# Autodesk Inventor assembly: 26650PACK
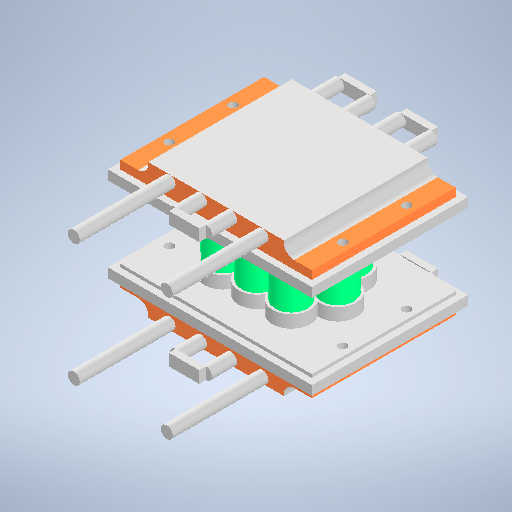
[picture p0: Inventor's stored thumbnail of the model, 512x512]
Saved by Autodesk Inventor 2025.2 (Build 292293000, 293)
## iProperties
Created: 2025-01-16
Part Number: 26650PACK
Document SubType Name: Assembly
Designer: cbast
Author: cbast
## Documents named in this file (6)
- C:\Users\cbast\OneDrive\Documents\26650PACK.iam
- C:\Users\cbast\OneDrive\Documents\26650(Green).ipt
- C:\Users\cbast\OneDrive\Documents\CELLCASE26650.ipt
- C:\Users\cbast\OneDrive\Documents\nickel strip.ipt
- C:\Users\cbast\OneDrive\Documents\cooling plate.ipt
- C:\Users\cbast\OneDrive\Documents\343thermalpad.ipt
## Components (18 placed, 5 different names)
1. 26650(Green):1 — Mate:2, Flush:2
2. 26650(Green):2 — Mate:1, Flush:1
3. 26650(Green):3 — Mate:3, Flush:3
4. 26650(Green):4 — Mate:4, Flush:7, Mate:12, Flush:11
5. 26650(Green):5 — Mate:5, Flush:6
6. 26650(Green):6 — Mate:10, Flush:8
7. 26650(Green):7 — Mate:9, Flush:9
8. 26650(Green):8 — Mate:8, Flush:10
9. 26650(Green):9 — Mate:7, Flush:4, Mate:11
10. 26650(Green):10 — Mate:6, Flush:5
11. CELLCASE26650:1 — Mate:1, Mate:2, Mate:3, Mate:4, Mate:5, Mate:6, Mate:7, Mate:8, Mate:9, Mate:10, Flush:1, Flush:2, Flush:3, Flush:4, Flush:5, Flush:6, Flush:7, Flush:8, Flush:9, Flush:10, Mate:13, Mate:22, Mate:23
12. CELLCASE26650:2 — Mate:11, Mate:12, Flush:11, Mate:15, Mate:18, Mate:19, Mate:20
13. 343thermalpad:1 — Mate:16, Mate:17
14. 343thermalpad:2 — Mate:14, Mate:21
15. nickel strip:1 — Mate:15, Mate:16
16. nickel strip:2 — Mate:13, Mate:14
17. cooling plate:1 — Mate:21, Mate:22, Mate:23
18. cooling plate:2 — Mate:17, Mate:18, Mate:19, Mate:20
## Relationships (34: Mate 23, Flush 11)
- Mate:1: 26650(Green):2 ↔ CELLCASE26650:1
- Mate:2: 26650(Green):1 ↔ CELLCASE26650:1
- Mate:3: 26650(Green):3 ↔ CELLCASE26650:1
- Mate:4: 26650(Green):4 ↔ CELLCASE26650:1
- Mate:5: 26650(Green):5 ↔ CELLCASE26650:1
- Mate:6: 26650(Green):10 ↔ CELLCASE26650:1
- Mate:7: 26650(Green):9 ↔ CELLCASE26650:1
- Mate:8: 26650(Green):8 ↔ CELLCASE26650:1
- Mate:9: 26650(Green):7 ↔ CELLCASE26650:1
- Mate:10: 26650(Green):6 ↔ CELLCASE26650:1
- Flush:1: 26650(Green):2 ↔ CELLCASE26650:1
- Flush:2: 26650(Green):1 ↔ CELLCASE26650:1
- Flush:3: 26650(Green):3 ↔ CELLCASE26650:1
- Flush:4: 26650(Green):9 ↔ CELLCASE26650:1
- Flush:5: 26650(Green):10 ↔ CELLCASE26650:1
- Flush:6: 26650(Green):5 ↔ CELLCASE26650:1
- Flush:7: 26650(Green):4 ↔ CELLCASE26650:1
- Flush:8: 26650(Green):6 ↔ CELLCASE26650:1
- Flush:9: 26650(Green):7 ↔ CELLCASE26650:1
- Flush:10: 26650(Green):8 ↔ CELLCASE26650:1
- Mate:11: 26650(Green):9 ↔ CELLCASE26650:2
- Mate:12: 26650(Green):4 ↔ CELLCASE26650:2
- Flush:11: 26650(Green):4 ↔ CELLCASE26650:2
- Mate:13: CELLCASE26650:1 ↔ nickel strip:2
- Mate:14: 343thermalpad:2 ↔ nickel strip:2
- Mate:15: CELLCASE26650:2 ↔ nickel strip:1
- Mate:16: 343thermalpad:1 ↔ nickel strip:1
- Mate:17: 343thermalpad:1 ↔ cooling plate:2
- Mate:18: CELLCASE26650:2 ↔ cooling plate:2
- Mate:19: CELLCASE26650:2 ↔ cooling plate:2
- Mate:20: CELLCASE26650:2 ↔ cooling plate:2
- Mate:21: 343thermalpad:2 ↔ cooling plate:1
- Mate:22: CELLCASE26650:1 ↔ cooling plate:1
- Mate:23: CELLCASE26650:1 ↔ cooling plate:1
